# Autodesk Inventor assembly: 01_light_wheel
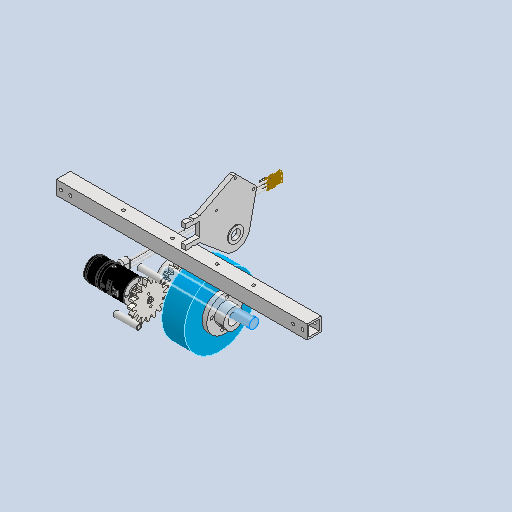
[picture p0: Inventor's stored thumbnail of the model, 512x512]
Saved by Autodesk Inventor 2025.2 (Build 292293000, 293)
## iProperties
Created: 2025-05-05
Part Number: 01_light_wheel
Document SubType Name: Assembly
Designer: yuki0520
Author: yuki0520
## Documents named in this file (15)
- C:\Users\haruy\Documents\ロボコン\NHK2025\cad\nagahisa\tanaka_dribll\2025_nhk\01\01_light_wheel.iam
- C:\Users\haruy\Documents\ロボコン\NHK2025\cad\nagahisa\tanaka_dribll\2025_nhk\01\light_kaku_2020.ipt
- C:\Users\haruy\Documents\ロボコン\NHK2025\cad\nagahisa\tanaka_dribll\2025_nhk\01\light_plate_middle.ipt
- C:\Users\haruy\Documents\ロボコン\NHK2025\cad\nagahisa\tanaka_dribll\2025_nhk\01\light_plate_motor.ipt
- C:\Users\haruy\Documents\ロボコン\NHK2025\cad\nagahisa\tanaka_dribll\2025_nhk\01\light_plate_nomo.ipt
- C:\Users\haruy\Documents\ロボコン\NHK2025\cad\000_parts\モーター\robomaster\M2006 P36\RoboMaster M2006 P36\RoboMaster M2006 P36.ipt
- C:\Users\haruy\Documents\ロボコン\NHK2025\cad\nagahisa\tanaka_dribll\2025_nhk\tanaka\nageru\smallring\small_tire.ipt
- C:\Users\haruy\Documents\ロボコン\NHK2025\cad\nagahisa\tanaka_dribll\2025_nhk\01\light_bar_roller_10.ipt
- C:\Users\haruy\Documents\ロボコン\NHK2025\cad\nagahisa\tanaka_dribll\2025_nhk\01\light_tire_fixer_10.ipt
- C:\Users\haruy\Documents\ロボコン\NHK2025\cad\nagahisa\tanaka_dribll\2025_nhk\01\light_gear.iam
- C:\Users\haruy\Documents\ロボコン\NHK2025\cad\nagahisa\tanaka_dribll\2025_nhk\01\set_6_20.ipt
- C:\Users\haruy\Documents\ロボコン\NHK2025\cad\nagahisa\tanaka_dribll\2025_nhk\01\light_space_6.ipt
- C:\Users\haruy\Documents\ロボコン\NHK2025\cad\nagahisa\tanaka_dribll\2025_nhk\01\set_bear_10.ipt
- C:\Users\haruy\Documents\ロボコン\NHK2025\cad\nagahisa\tanaka_dribll\2025_nhk\01\set_10_28.ipt
- C:\Users\haruy\Documents\ロボコン\NHK2025\cad\000_parts\ベアリング\10\bear_10_15_sn.ipt
## Components (16 placed, 14 different names)
1. light_kaku_2020:1 — メイト:37
2. light_plate_middle:1
3. light_plate_motor:1
4. light_plate_nomo:1 — 挿入:18
5. RoboMaster M2006 P36:1 — メイト:35
6. small_tire:1 — 挿入:5, 挿入:6
7. light_bar_roller_10:1 — メイト:30, メイト:34, メイト:39
8. light_tire_fixer_10:2 — 挿入:5, 挿入:6, メイト:30
9. light_gear:1 [sub-assembly] — メイト:34, メイト:35, 挿入:7, 挿入:8, 挿入:16, 挿入:17
10. set_6_20:1 — 挿入:7, 挿入:8
11. light_space_6:1
12. light_space_6:2
13. light_space_6:3
14. set_bear_10:1 — メイト:39
15. set_10_28:1 — 挿入:16, 挿入:17
16. bear_10_15_sn:1 — 挿入:18
## Relationships (12: Insert 7, Mate 5)
- 挿入:5 [Insert]: small_tire:1 ↔ light_tire_fixer_10:2
- 挿入:6 [Insert]: small_tire:1 ↔ light_tire_fixer_10:2
- メイト:30 [Mate]: light_bar_roller_10:1 ↔ light_tire_fixer_10:2
- メイト:34 [Mate]: light_bar_roller_10:1 ↔ light_gear:1
- メイト:35 [Mate]: RoboMaster M2006 P36:1 ↔ light_gear:1
- 挿入:7 [Insert]: light_gear:1 ↔ set_6_20:1
- 挿入:8 [Insert]: light_gear:1 ↔ set_6_20:1
- メイト:37 [Mate]: light_kaku_2020:1
- メイト:39 [Mate]: light_bar_roller_10:1 ↔ set_bear_10:1
- 挿入:16 [Insert]: light_gear:1 ↔ set_10_28:1
- 挿入:17 [Insert]: light_gear:1 ↔ set_10_28:1
- 挿入:18 [Insert]: light_plate_nomo:1 ↔ bear_10_15_sn:1
